# Autodesk Inventor assembly: 22nc_plate3_motor
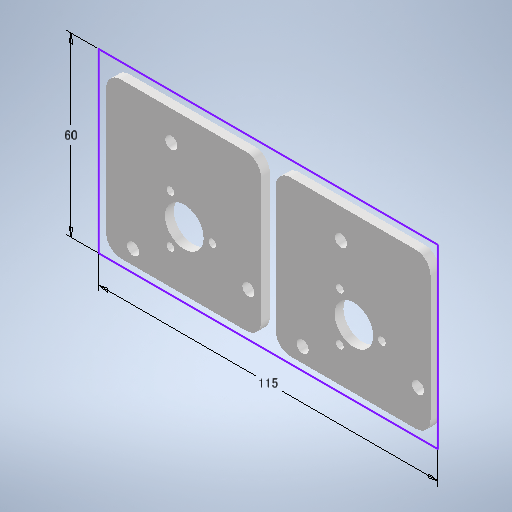
[picture p0: Inventor's stored thumbnail of the model, 512x512]
Saved by Autodesk Inventor 2025.1 (Build 291241000, 241)
## iProperties
Created: 2025-05-06
Part Number: 22nc_plate3_motor
Document SubType Name: Assembly
Designer: yuki0520
Author: yuki0520
## Documents named in this file (2)
- C:\Users\yuki0520\OneDrive\ドキュメント\Inventor\2025_nhk\tanaka\nageru\light\22nc_plate3_motor.iam
- C:\Users\yuki0520\OneDrive\ドキュメント\Inventor\2025_nhk\tanaka\nageru\light\light_plate_motor.ipt
## Components (2 placed, 1 different names)
1. light_plate_motor:1 — フラッシュ:1, メイト:1, フラッシュ:2
2. light_plate_motor:2 — フラッシュ:1, メイト:1, フラッシュ:2
## Relationships (3: Flush 2, Mate 1)
- フラッシュ:1 [Flush]: light_plate_motor:1 ↔ light_plate_motor:2
- メイト:1 [Mate] (5 mm): light_plate_motor:1 ↔ light_plate_motor:2
- フラッシュ:2 [Flush]: light_plate_motor:1 ↔ light_plate_motor:2
